# Autodesk Inventor assembly: Assembly1
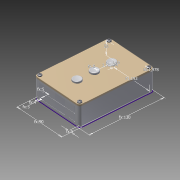
[picture p0: Inventor's stored thumbnail of the model, 180x180]
Saved by Autodesk Inventor 2013 (Build 170138000, 138)
## iProperties
Created: 2013-01-11
Part Number: Assembly1
Document SubType Name: Assembly
Designer: md
Author: md
## Documents named in this file (6)
- X:\Projects\hexasense\enclosure\sense_board\Assembly1.iam
- X:\Projects\hexasense\enclosure\sense_board\frontplatte.ipt
- X:\Projects\hexasense\enclosure\sense_board\pushbutton.ipt
- X:\Projects\hexasense\enclosure\sense_board\PCB-Model.ipt
- X:\Projects\hexasense\enclosure\sense_board\base.ipt
- C:\Users\md\Documents\Inventor\Content Center Files\R2013\en-US\ISO 7049 - C-Z(2)\ISO 7049 - ST 3,5 x 9,5 - C - Z.ipt
## Components (13 placed, 5 different names)
1. frontplatte:1 — Insert:6, Insert:7, Mate:1, Insert:8, Insert:9, Insert:10, Insert:11
2. pushbutton:1 — Insert:2
3. pushbutton:2 — Insert:3
4. pushbutton:3 — Insert:1
5. PCB-Model:1 — Insert:1, Insert:2, Insert:3, Insert:12, Insert:13, Insert:15
6. base:1 — Insert:6, Insert:7, Mate:1
7. ISO 7049 - C-Z ST 3,5 x 9,5 - C - Z:1 — Insert:8
8. ISO 7049 - C-Z ST 3,5 x 9,5 - C - Z:2 — Insert:9
9. ISO 7049 - C-Z ST 3,5 x 9,5 - C - Z:3 — Insert:10
10. ISO 7049 - C-Z ST 3,5 x 9,5 - C - Z:4 — Insert:11
11. ISO 7049 - C-Z ST 3,5 x 9,5 - C - Z:5 — Insert:12
12. ISO 7049 - C-Z ST 3,5 x 9,5 - C - Z:6 — Insert:13
13. ISO 7049 - C-Z ST 3,5 x 9,5 - C - Z:8 — Insert:15
## Relationships (13: Insert 12, Mate 1)
- Insert:1 (-5 mm): pushbutton:3 ↔ PCB-Model:1
- Insert:2 (-5 mm): pushbutton:1 ↔ PCB-Model:1
- Insert:3 (-5 mm): pushbutton:2 ↔ PCB-Model:1
- Insert:6: frontplatte:1 ↔ base:1
- Insert:7: frontplatte:1 ↔ base:1
- Mate:1: frontplatte:1 ↔ base:1
- Insert:8: frontplatte:1 ↔ ISO 7049 - C-Z ST 3,5 x 9,5 - C - Z:1
- Insert:9: frontplatte:1 ↔ ISO 7049 - C-Z ST 3,5 x 9,5 - C - Z:2
- Insert:10: frontplatte:1 ↔ ISO 7049 - C-Z ST 3,5 x 9,5 - C - Z:3
- Insert:11: frontplatte:1 ↔ ISO 7049 - C-Z ST 3,5 x 9,5 - C - Z:4
- Insert:12: PCB-Model:1 ↔ ISO 7049 - C-Z ST 3,5 x 9,5 - C - Z:5
- Insert:13: PCB-Model:1 ↔ ISO 7049 - C-Z ST 3,5 x 9,5 - C - Z:6
- Insert:15: PCB-Model:1 ↔ ISO 7049 - C-Z ST 3,5 x 9,5 - C - Z:8
